# Autodesk Inventor assembly: ASY MSC 002 отстойник осветлитель
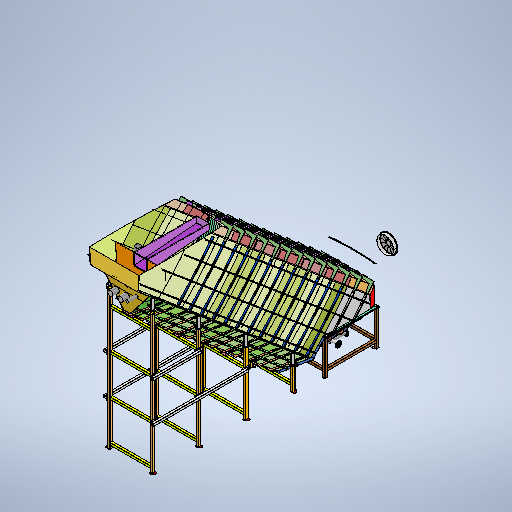
[picture p0: Inventor's stored thumbnail of the model, 512x512]
Saved by Autodesk Inventor 2025 (Build 290162010, 162A)
## iProperties
Created: 2024-09-05
Part Number: ASY MSC 002 отстойник осветлитель
Document SubType Name: Assembly
Designer: admin
Author: admin
## Documents named in this file (39)
- C:\Users\admin\YandexDisk-badmisterfox\домашниий пк\Inventor\Manturovo\Manturovo_Se-clar\ASY MSC 002 отстойник осветлитель.iam
- C:\Users\admin\YandexDisk-badmisterfox\домашниий пк\Inventor\Manturovo\Manturovo_Se-clar\ASY MSC 900.1 base frame.iam
- C:\Users\admin\YandexDisk-badmisterfox\домашниий пк\Inventor\Manturovo\Manturovo_Se-clar\ASY MSC 100 cone.iam
- C:\Users\admin\YandexDisk-badmisterfox\домашниий пк\Inventor\Manturovo\Manturovo_Se-clar\MSC 401 sheet lowerback.ipt
- C:\Users\admin\YandexDisk-badmisterfox\домашниий пк\Inventor\Manturovo\Manturovo_Se-clar\MSC 706 ridge 1.ipt
- C:\Users\admin\YandexDisk-badmisterfox\домашниий пк\Inventor\Manturovo\Manturovo_Se-clar\MSC 701 face 1.ipt
- C:\Users\admin\YandexDisk-badmisterfox\домашниий пк\Inventor\Manturovo\Manturovo_Se-clar\MSC 705 ridge 3.ipt
- C:\Users\admin\YandexDisk-badmisterfox\домашниий пк\Inventor\Manturovo\Manturovo_Se-clar\MSC 713 tube.ipt
- C:\Users\admin\YandexDisk-badmisterfox\домашниий пк\Inventor\Manturovo\Manturovo_Se-clar\ISO 5251 Bends 3D without straight ends(90 deg) DN150 11 11.ipt
- C:\Users\admin\YandexDisk-badmisterfox\домашниий пк\Inventor\Manturovo\Manturovo_Se-clar\MSC 712 tube.ipt
- C:\Users\admin\YandexDisk-badmisterfox\домашниий пк\Inventor\Manturovo\Manturovo_Se-clar\MSC 711 tube.ipt
- C:\Users\admin\YandexDisk-badmisterfox\домашниий пк\Inventor\Manturovo\Manturovo_Se-clar\MSC 408 stringer lowerback.ipt
- C:\Users\admin\YandexDisk-badmisterfox\домашниий пк\Inventor\Manturovo\Manturovo_Se-clar\MSC 707 ridge 2.ipt
- C:\Users\admin\YandexDisk-badmisterfox\домашниий пк\Inventor\Manturovo\Manturovo_Se-clar\MSC 703 face 2.ipt
- C:\Users\admin\YandexDisk-badmisterfox\домашниий пк\Inventor\Manturovo\Manturovo_Se-clar\MSC 702 face 3.ipt
- C:\Users\admin\YandexDisk-badmisterfox\домашниий пк\Inventor\Manturovo\Manturovo_Se-clar\MSC 704 face 4.ipt
- C:\Users\admin\YandexDisk-badmisterfox\домашниий пк\Inventor\Manturovo\Manturovo_Se-clar\MSC 708 ridge 4.ipt
- C:\Users\admin\YandexDisk-badmisterfox\домашниий пк\Inventor\Manturovo\Manturovo_Se-clar\MSC 709 ridge 5.ipt
- C:\Users\admin\YandexDisk-badmisterfox\домашниий пк\Inventor\Manturovo\Manturovo_Se-clar\ASY MSC 900.3 base frame.iam
- C:\Users\admin\YandexDisk-badmisterfox\домашниий пк\Inventor\Manturovo\Manturovo_Se-clar\Pillars\ASY MSC 900.5 base frame.iam
- C:\Users\admin\YandexDisk-badmisterfox\домашниий пк\Inventor\Manturovo\Manturovo_Se-clar\Pillars\ASY MSC 900.4  base frame.iam
- C:\Users\admin\YandexDisk-badmisterfox\домашниий пк\Inventor\Manturovo\Manturovo_Se-clar\Pillars\ASY MSC 900.6 base frame.iam
- C:\Users\admin\YandexDisk-badmisterfox\домашниий пк\Inventor\Manturovo\Manturovo_Se-clar\ASY MSC 200 BACK.iam
- C:\Users\admin\YandexDisk-badmisterfox\домашниий пк\Inventor\Manturovo\Manturovo_Se-clar\ASY MSC 300.2 LEFT BOARD.iam
- C:\Users\admin\YandexDisk-badmisterfox\домашниий пк\Inventor\Manturovo\Manturovo_Se-clar\ASY MSC 300.1 RIGHT BOARD.iam
- C:\Users\admin\YandexDisk-badmisterfox\домашниий пк\Inventor\Manturovo\Manturovo_Se-clar\ASY MSC 500 BELLY.iam
- C:\Users\admin\YandexDisk-badmisterfox\домашниий пк\Inventor\Manturovo\Manturovo_Se-clar\ASY MSC 900.2 support.iam
- C:\Users\admin\YandexDisk-badmisterfox\домашниий пк\Inventor\Manturovo\Manturovo_Se-clar\ASY MSC 600 cone exit back.iam
- C:\Users\admin\YandexDisk-badmisterfox\домашниий пк\Inventor\Manturovo\Manturovo_Se-clar\ASY MSC 800 gills.iam
- C:\Users\admin\YandexDisk-badmisterfox\домашниий пк\Inventor\Manturovo\Manturovo_Se-clar\MSC 407 sheet lowerback_FIX.ipt
- C:\Users\admin\YandexDisk-badmisterfox\домашниий пк\Inventor\Manturovo\Manturovo_Se-clar\ASY MSC 400 Accsess hatch.iam
- C:\Users\admin\YandexDisk-badmisterfox\домашниий пк\Inventor\Manturovo\Manturovo_Se-clar\MSC DIM 000 settler-clarifier.ipt
- C:\Users\admin\YandexDisk-badmisterfox\домашниий пк\Inventor\Manturovo\Manturovo_Se-clar\MSC DIM 001 frame.ipt
- C:\Users\admin\YandexDisk-badmisterfox\домашниий пк\Inventor\Manturovo\Manturovo_Se-clar\ASY MSC 900.7 base frame transverse.iam
- C:\Users\admin\YandexDisk-badmisterfox\домашниий пк\Inventor\Manturovo\Manturovo_Se-clar\ASY MSC 900.8 base frame transverse.iam
- C:\Users\admin\YandexDisk-badmisterfox\домашниий пк\Inventor\Manturovo\Manturovo_Se-clar\ASY MSC 900.8 base frame transverse.ipt
- C:\Users\admin\YandexDisk-badmisterfox\домашниий пк\Inventor\Manturovo\Manturovo_Se-clar\ISO 657_14 - 60x40x3 - 1000.ipt
- C:\Users\admin\YandexDisk-badmisterfox\домашниий пк\Inventor\Manturovo\Manturovo_Se-clar\Part2.ipt
- C:\Users\admin\YandexDisk-badmisterfox\домашниий пк\Inventor\Manturovo\Manturovo_Se-clar\MSC 900.9 base frame transverse.ipt
## Components (58 placed, 38 different names)
1. MSC DIM 000 settler-clarifier.ipt:1
2. MSC DIM 001 frame.ipt:1
3. ASY MSC 900.1 base frame.iam:1 [sub-assembly] — Flush:4, Mate:18, Flush:5, Mate:19, Mate:44, Mate:47, Mate:50, Mate:66, Flush:16
4. ASY MSC 100 cone.iam:1 [sub-assembly] — Mate:19, Flush:6, Mate:29, Rigid:17
5. MSC 401 sheet lowerback.ipt:1 — Mate:29, Mate:30, Mate:31
6. MSC 706 ridge 1.ipt:1
7. MSC 701 face 1.ipt:1 — Flush:9, Mate:35
8. MSC 705 ridge 3.ipt:1 — Rigid:12, Rigid:14
9. MSC 713 tube.ipt:1
10. ISO 5251 Bends 3D without straight ends(90 deg) DN150 11 11.ipt:1
11. MSC 712 tube.ipt:1
12. MSC 711 tube.ipt:1
13. MSC 408 stringer lowerback.ipt:1
14. MSC 707 ridge 2.ipt:1 — Rigid:12, Rigid:13
15. MSC 713 tube.ipt:2
16. MSC 703 face 2.ipt:1 — Mate:37, Flush:12, Flush:13
17. MSC 702 face 3.ipt:1 — Mate:34, Mate:35, Mate:36
18. MSC 704 face 4.ipt:1
19. MSC 408 stringer lowerback.ipt:2
20. MSC 708 ridge 4.ipt:1 — Rigid:14
21. MSC 709 ridge 5.ipt:1 — Rigid:13
22. ASY MSC 900.3 base frame.iam:1 [sub-assembly] — Mate:23, Mate:24, Cylindrical:4, Mate:44, Mate:45, Mate:49, Flush:14, Rigid:26
23. ASY MSC 900.5 base frame.iam:1 [sub-assembly] — Flush:11, Cylindrical:7, Cylindrical:8, Mate:46, Mate:48, Rigid:28
24. ASY MSC 900.4  base frame.iam:1 [sub-assembly] — Mate:32, Mate:33, Mate:45, Mate:46, Rigid:27
25. ASY MSC 900.6 base frame.iam:1 [sub-assembly] — Mate:38, Mate:39, Cylindrical:5, Cylindrical:6, Mate:47, Rigid:19, Rigid:20, Rigid:21, Rigid:22, Rigid:29
26. ASY MSC 200 BACK.iam:1 [sub-assembly] — Flush:8, Mate:31
27. ASY MSC 300.2 LEFT BOARD.iam:1 [sub-assembly] — Rigid:11, Mate:34, Flush:12
28. ASY MSC 300.1 RIGHT BOARD.iam:1 [sub-assembly] — Rigid:10, Mate:37
29. ASY MSC 500 BELLY.iam:1 [sub-assembly] — Flush:7, Mate:22, Mate:25, Rigid:10, Rigid:11, Mate:40, Mate:41, Mate:42, Mate:43
30. ASY MSC 900.2 support.iam:1 [sub-assembly] — Cylindrical:8, Mate:40
31. ASY MSC 900.2 support.iam:2 [sub-assembly]
32. ASY MSC 900.2 support.iam:3 [sub-assembly] — Cylindrical:4, Mate:25
33. ASY MSC 900.2 support.iam:4 [sub-assembly] — Cylindrical:6, Mate:42
34. ASY MSC 900.2 support.iam:5 [sub-assembly]
35. ASY MSC 600 cone exit back.iam:1 [sub-assembly] — Rigid:17
36. ASY MSC 800 gills.iam:1 [sub-assembly] — Mate:22
37. MSC 407 sheet lowerback_FIX.ipt:1
38. ASY MSC 900.2 support.iam:6 [sub-assembly] — Cylindrical:7, Mate:41
39. ASY MSC 900.2 support.iam:7 [sub-assembly]
40. ASY MSC 400 Accsess hatch.iam:1 [sub-assembly]
41. ASY MSC 900.2 support.iam:8 [sub-assembly] — Cylindrical:5, Mate:43
42. ASY MSC 900.7 base frame transverse.iam:1 [sub-assembly] — Rigid:19
43. ASY MSC 900.7 base frame transverse.iam:2 [sub-assembly] — Rigid:20
44. ASY MSC 900.8 base frame transverse.iam:1 [sub-assembly] — Rigid:21
45. ASY MSC 900.8 base frame transverse.iam:2 [sub-assembly] — Rigid:22
46. ASY MSC 900.8 base frame transverse:3 — Rigid:23, Flush:15
47. ASY MSC 900.8 base frame transverse:4 — Rigid:23, Mate:50, Mate:66, Flush:16
48. ASY MSC 900.8 base frame transverse:5 — Rigid:24, Rigid:25
49. ASY MSC 900.8 base frame transverse:6 — Rigid:24, Mate:49, Flush:14, Flush:15
50. ISO 657_14 - 60x40x3 - 1000:1 — Rigid:25
51. Part2:1 — Rigid:26, Mate:51, Mate:52
52. MSC 900.9 base frame transverse:1 — Mate:51, Mate:52
53. Part2:2 — Rigid:27, Mate:59
54. MSC 900.9 base frame transverse:2 — Mate:59
55. Part2:3 — Rigid:28
56. MSC 900.9 base frame transverse:3
57. Part2:4 — Rigid:29
58. MSC 900.9 base frame transverse:4
## Relationships (97: Mate 51, WeldJoint 22, Flush 15, CylindricalJoint 8, RevoluteJoint 1)
- [Mate]: ASY MSC 100 cone.iam:1 ↔ MSC 401 sheet lowerback.ipt:1
- [WeldJoint]: MSC 713 tube.ipt:1 ↔ ISO 5251 Bends 3D without straight ends(90 deg) DN150 11 11.ipt:1
- [Mate]: ASY MSC 100 cone.iam:1 ↔ MSC 408 stringer lowerback.ipt:1
- [RevoluteJoint]: ISO 5251 Bends 3D without straight ends(90 deg) DN150 11 11.ipt:1 ↔ MSC 713 tube.ipt:2
- [WeldJoint]: MSC 701 face 1.ipt:1 ↔ MSC 712 tube.ipt:1
- [WeldJoint]: MSC 701 face 1.ipt:1 ↔ MSC 711 tube.ipt:1
- [WeldJoint] (-200 mm): MSC 701 face 1.ipt:1 ↔ MSC 713 tube.ipt:1
- [Mate]: ASY MSC 100 cone.iam:1 ↔ MSC 408 stringer lowerback.ipt:2
- [Mate]: ASY MSC 500 BELLY.iam:1 ↔ ASY MSC 600 cone exit back.iam:1
- [Flush]: ASY MSC 900.1 base frame.iam:1 ↔ ASY MSC 100 cone.iam:1
- Rigid:12 [WeldJoint]: MSC 705 ridge 3.ipt:1 ↔ MSC 707 ridge 2.ipt:1
- [WeldJoint]: MSC 706 ridge 1.ipt:1 ↔ MSC 705 ridge 3.ipt:1
- [Flush]: ASY MSC 500 BELLY.iam:1 ↔ ASY MSC 600 cone exit back.iam:1
- [Mate]: ASY MSC 500 BELLY.iam:1 ↔ ASY MSC 800 gills.iam:1
- [Mate]: MSC 701 face 1.ipt:1 ↔ ASY MSC 500 BELLY.iam:1
- [Mate] (-5 mm): MSC 701 face 1.ipt:1 ↔ ASY MSC 500 BELLY.iam:1
- [Mate]: ASY MSC 500 BELLY.iam:1 ↔ ASY MSC 900.2 support.iam:2
- [Mate]: ASY MSC 500 BELLY.iam:1 ↔ ASY MSC 900.2 support.iam:5
- [Mate]: ASY MSC 500 BELLY.iam:1 ↔ ASY MSC 900.2 support.iam:7
- [CylindricalJoint]: ASY MSC 900.4  base frame.iam:1 ↔ ASY MSC 900.2 support.iam:5
- [CylindricalJoint]: ASY MSC 900.4  base frame.iam:1 ↔ ASY MSC 900.2 support.iam:2
- [Mate] (-2860 mm): ASY MSC 200 BACK.iam:1 ↔ ASY MSC 500 BELLY.iam:1
- [CylindricalJoint]: ASY MSC 900.3 base frame.iam:1 ↔ ASY MSC 900.2 support.iam:7
- [Flush]: ASY MSC 900.3 base frame.iam:1 ↔ ASY MSC 900.4  base frame.iam:1
- Flush:4: ASY MSC 900.1 base frame.iam:1
- Mate:18 (4 mm): ASY MSC 900.1 base frame.iam:1
- Flush:5: ASY MSC 900.1 base frame.iam:1
- Mate:19: ASY MSC 900.1 base frame.iam:1 ↔ ASY MSC 100 cone.iam:1
- Flush:6: ASY MSC 100 cone.iam:1
- Flush:7: ASY MSC 500 BELLY.iam:1
- Flush:8: ASY MSC 200 BACK.iam:1
- Mate:22: ASY MSC 500 BELLY.iam:1 ↔ ASY MSC 800 gills.iam:1
- Mate:23: ASY MSC 900.3 base frame.iam:1
- Mate:24: ASY MSC 900.3 base frame.iam:1
- Cylindrical:4: ASY MSC 900.3 base frame.iam:1 ↔ ASY MSC 900.2 support.iam:3
- Mate:25: ASY MSC 500 BELLY.iam:1 ↔ ASY MSC 900.2 support.iam:3
- Flush:9: MSC 701 face 1.ipt:1
- Mate:29: ASY MSC 100 cone.iam:1 ↔ MSC 401 sheet lowerback.ipt:1
- Mate:30: MSC 401 sheet lowerback.ipt:1
- Mate:31: MSC 401 sheet lowerback.ipt:1 ↔ ASY MSC 200 BACK.iam:1
- Rigid:10 [WeldJoint] (-25 mm): ASY MSC 300.1 RIGHT BOARD.iam:1 ↔ ASY MSC 500 BELLY.iam:1
- Rigid:11 [WeldJoint] (-25 mm): ASY MSC 300.2 LEFT BOARD.iam:1 ↔ ASY MSC 500 BELLY.iam:1
- Flush:11: ASY MSC 900.5 base frame.iam:1
- Mate:32: ASY MSC 900.4  base frame.iam:1
- Mate:33: ASY MSC 900.4  base frame.iam:1
- Mate:34: MSC 702 face 3.ipt:1 ↔ ASY MSC 300.2 LEFT BOARD.iam:1
- Mate:35: MSC 701 face 1.ipt:1 ↔ MSC 702 face 3.ipt:1
- Rigid:13 [WeldJoint]: MSC 707 ridge 2.ipt:1 ↔ MSC 709 ridge 5.ipt:1
- Rigid:14 [WeldJoint]: MSC 705 ridge 3.ipt:1 ↔ MSC 708 ridge 4.ipt:1
- Mate:36: MSC 702 face 3.ipt:1
- Mate:37: MSC 703 face 2.ipt:1 ↔ ASY MSC 300.1 RIGHT BOARD.iam:1
- Mate:38: ASY MSC 900.6 base frame.iam:1
- Mate:39: ASY MSC 900.6 base frame.iam:1
- Cylindrical:5: ASY MSC 900.6 base frame.iam:1 ↔ ASY MSC 900.2 support.iam:8
- Cylindrical:6: ASY MSC 900.6 base frame.iam:1 ↔ ASY MSC 900.2 support.iam:4
- Cylindrical:7: ASY MSC 900.5 base frame.iam:1 ↔ ASY MSC 900.2 support.iam:6
- Cylindrical:8: ASY MSC 900.5 base frame.iam:1 ↔ ASY MSC 900.2 support.iam:1
- Mate:40 (3 mm): ASY MSC 500 BELLY.iam:1 ↔ ASY MSC 900.2 support.iam:1
- Mate:41 (3 mm): ASY MSC 500 BELLY.iam:1 ↔ ASY MSC 900.2 support.iam:6
- Mate:42: ASY MSC 500 BELLY.iam:1 ↔ ASY MSC 900.2 support.iam:4
- Mate:43: ASY MSC 500 BELLY.iam:1 ↔ ASY MSC 900.2 support.iam:8
- Flush:12: MSC 703 face 2.ipt:1 ↔ ASY MSC 300.2 LEFT BOARD.iam:1
- Flush:13: MSC 703 face 2.ipt:1
- Mate:44 (820 mm): ASY MSC 900.1 base frame.iam:1 ↔ ASY MSC 900.3 base frame.iam:1
- Mate:45 (1430 mm): ASY MSC 900.3 base frame.iam:1 ↔ ASY MSC 900.4  base frame.iam:1
- Mate:46 (1430 mm): ASY MSC 900.5 base frame.iam:1 ↔ ASY MSC 900.4  base frame.iam:1
- Mate:47 (5315 mm): ASY MSC 900.1 base frame.iam:1 ↔ ASY MSC 900.6 base frame.iam:1
- Rigid:17 [WeldJoint]: ASY MSC 100 cone.iam:1 ↔ ASY MSC 600 cone exit back.iam:1
- Mate:48: ASY MSC 900.5 base frame.iam:1
- Rigid:19 [WeldJoint]: ASY MSC 900.6 base frame.iam:1 ↔ ASY MSC 900.7 base frame transverse.iam:1
- Rigid:20 [WeldJoint]: ASY MSC 900.6 base frame.iam:1 ↔ ASY MSC 900.7 base frame transverse.iam:2
- Rigid:21 [WeldJoint]: ASY MSC 900.6 base frame.iam:1 ↔ ASY MSC 900.8 base frame transverse.iam:1
- Rigid:22 [WeldJoint]: ASY MSC 900.6 base frame.iam:1 ↔ ASY MSC 900.8 base frame transverse.iam:2
- Rigid:23 [WeldJoint]: ASY MSC 900.8 base frame transverse:3 ↔ ASY MSC 900.8 base frame transverse:4
- Rigid:24 [WeldJoint]: ASY MSC 900.8 base frame transverse:5 ↔ ASY MSC 900.8 base frame transverse:6
- Mate:49: ASY MSC 900.3 base frame.iam:1 ↔ ASY MSC 900.8 base frame transverse:6
- Mate:50: ASY MSC 900.1 base frame.iam:1 ↔ ASY MSC 900.8 base frame transverse:4
- Flush:14 (-40 mm): ASY MSC 900.3 base frame.iam:1 ↔ ASY MSC 900.8 base frame transverse:6
- Flush:15: ASY MSC 900.8 base frame transverse:3 ↔ ASY MSC 900.8 base frame transverse:6
- Rigid:25 [WeldJoint]: ASY MSC 900.8 base frame transverse:5 ↔ ISO 657_14 - 60x40x3 - 1000:1
- Rigid:26 [WeldJoint]: ASY MSC 900.3 base frame.iam:1 ↔ Part2:1
- Mate:51: Part2:1 ↔ MSC 900.9 base frame transverse:1
- Mate:52 (-10 mm): Part2:1 ↔ MSC 900.9 base frame transverse:1
- [Mate]: Part2:2 ↔ MSC 900.9 base frame transverse:2
- [Mate] (-10 mm): Part2:2 ↔ MSC 900.9 base frame transverse:2
- Rigid:27 [WeldJoint]: ASY MSC 900.4  base frame.iam:1 ↔ Part2:2
- Mate:59: Part2:2 ↔ MSC 900.9 base frame transverse:2
- [Mate]: Part2:3 ↔ MSC 900.9 base frame transverse:3
- [Mate] (-10 mm): Part2:3 ↔ MSC 900.9 base frame transverse:3
- [Mate]: Part2:3 ↔ MSC 900.9 base frame transverse:3
- [Mate]: Part2:4 ↔ MSC 900.9 base frame transverse:4
- [Mate] (-10 mm): Part2:4 ↔ MSC 900.9 base frame transverse:4
- [Mate]: Part2:4 ↔ MSC 900.9 base frame transverse:4
- Rigid:28 [WeldJoint]: ASY MSC 900.5 base frame.iam:1 ↔ Part2:3
- Rigid:29 [WeldJoint]: ASY MSC 900.6 base frame.iam:1 ↔ Part2:4
- Mate:66: ASY MSC 900.1 base frame.iam:1 ↔ ASY MSC 900.8 base frame transverse:4
- Flush:16 (-40 mm): ASY MSC 900.1 base frame.iam:1 ↔ ASY MSC 900.8 base frame transverse:4
## Named parameters: d131_d129 = 0 mm, d132_d130 = -10 mm, d139_d131_d129 = 0 mm, d140_d132_d130 = -10 mm, d141_d138 = 0 mm, d142_d131_d129 = 0 mm, d143_d132_d130 = -10 mm, d144_d138 = 0 mm
